# Autodesk Inventor assembly: Ensamble final
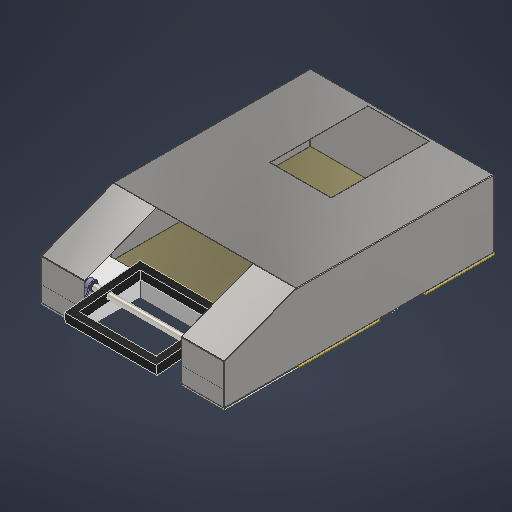
[picture p0: Inventor's stored thumbnail of the model, 512x512]
Saved by Autodesk Inventor 2026.3 (Build 303398000, 398)
## iProperties
Created: 2026-06-07
Part Number: Ensamble final
Document SubType Name: Assembly
Designer: user
Author: user
## Documents named in this file (8)
- C:\Users\user\Documents\Gabriel\Proyectos\Robot de pelea\Diseños Inventor\Diseño final\Ensamble final.iam
- C:\Users\user\Documents\Gabriel\Proyectos\Robot de pelea\Diseños Inventor\Part1.ipt
- C:\Users\user\Documents\Gabriel\Proyectos\Robot de pelea\Diseños Inventor\Part6.ipt
- C:\Users\user\Documents\Gabriel\Proyectos\Robot de pelea\Diseños Inventor\Part5.ipt
- C:\Users\user\Documents\Gabriel\Proyectos\Robot de pelea\Diseños Inventor\Part4.ipt
- C:\Users\user\Documents\Gabriel\Proyectos\Robot de pelea\Diseños Inventor\Diseño final\Carcasa.ipt
- C:\Users\user\Documents\Gabriel\Proyectos\Robot de pelea\Diseños Inventor\Diseño final\Part2.ipt
- C:\Users\user\Documents\Gabriel\Proyectos\Robot de pelea\Diseños Inventor\Diseño final\Arma\Ensamblaje arma.iam
## Components (10 placed, 7 different names)
1. Part1:2 — Mate:8, Mate:10, Flush:4, Mate:20, Flush:5, Flush:6, Flush:7, Flush:8
2. Part6:1 — Flush:3, Flush:4, Mate:12
3. Part6:2 — Mate:8, Mate:10, Flush:3, Mate:14
4. Part5:1 — Mate:12, Mate:16, Mate:19
5. Part5:2 — Mate:14, Mate:17, Mate:18
6. Part4:1 — Mate:17, Mate:18
7. Part4:2 — Mate:16, Mate:19
8. Carcasa:1 — Mate:20, Flush:5, Flush:6, Mate:22, Mate:23
9. Part2:1 — Flush:7, Flush:8, Mate:21
10. Ensamblaje arma:1 [sub-assembly] — Mate:21, Mate:22, Mate:23
## Relationships (18: Mate 12, Flush 6)
- Mate:8 (1 mm): Part1:2 ↔ Part6:2
- Mate:10 (7.25 mm): Part1:2 ↔ Part6:2
- Flush:3: Part6:1 ↔ Part6:2
- Flush:4 (-5 mm): Part1:2 ↔ Part6:1
- Mate:12: Part6:1 ↔ Part5:1
- Mate:14: Part6:2 ↔ Part5:2
- Mate:16: Part5:1 ↔ Part4:2
- Mate:17: Part5:2 ↔ Part4:1
- Mate:18: Part5:2 ↔ Part4:1
- Mate:19: Part5:1 ↔ Part4:2
- Mate:20: Part1:2 ↔ Carcasa:1
- Flush:5: Part1:2 ↔ Carcasa:1
- Flush:6: Part1:2 ↔ Carcasa:1
- Flush:7: Part1:2 ↔ Part2:1
- Flush:8: Part1:2 ↔ Part2:1
- Mate:21: Part2:1 ↔ Ensamblaje arma:1
- Mate:22 (14 mm): Carcasa:1 ↔ Ensamblaje arma:1
- Mate:23 (10 mm): Carcasa:1 ↔ Ensamblaje arma:1
